# Autodesk Inventor assembly: Mini Stealthburner
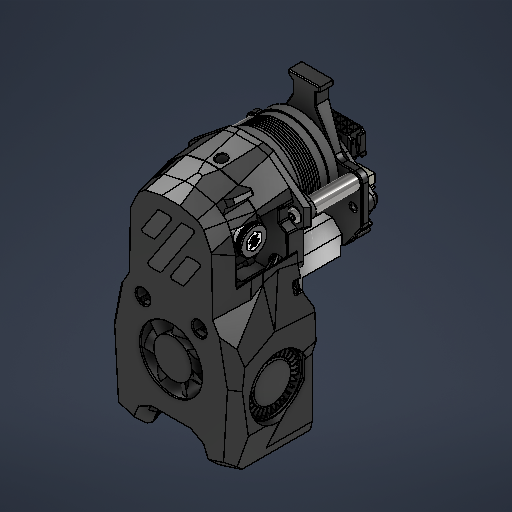
[picture p0: Inventor's stored thumbnail of the model, 512x512]
Saved by Autodesk Inventor 2026 (Build 300175050, 175E)
## iProperties
Created: 2025-05-09
Part Number: Mini Stealthburner
Document SubType Name: Assembly
Designer: AdminForWorker
Title: Mini Stealthburner
Author: AdminForWorker
## Documents named in this file (27)
- C:\Users\Joshua Eah\Documents\GitHub\Voron-0\CAD\Master Assembly\Toolhead\Mini Stealthburner.iam
- C:\Users\Joshua Eah\Documents\GitHub\Voron-0\CAD\Master Assembly\Toolhead\Parts\Extruder\36mm Round Stepper Motor.ipt
- C:\Users\Joshua Eah\Documents\GitHub\Voron-0\CAD\Master Assembly\Toolhead\Subassemblies\Hotend Assembly.iam
- C:\Users\Joshua Eah\Documents\GitHub\Voron-0\CAD\Master Assembly\Toolhead\Subassemblies\Front Cowling.iam
- C:\Users\Joshua Eah\Documents\GitHub\Voron-0\CAD\Machined Parts\X Carriage\X Carriage Body.ipt
- C:\Users\Joshua Eah\Documents\GitHub\Voron-0\CAD\Master Assembly\Hardware\M3x8 FHCS.ipt
- C:\Users\Joshua Eah\Documents\GitHub\Voron-0\CAD\Master Assembly\Hardware\M2x6 SHCS.ipt
- C:\Users\Joshua Eah\Documents\GitHub\Voron-0\CAD\Master Assembly\Hardware\M3x6 BHCS.ipt
- C:\Users\Joshua Eah\Documents\GitHub\Voron-0\CAD\Master Assembly\Hardware\M3x8 BHCS.ipt
- C:\Users\Joshua Eah\Documents\GitHub\Voron-0\CAD\Master Assembly\Hardware\M3x10 BHCS.ipt
- C:\Users\Joshua Eah\Documents\GitHub\Voron-0\CAD\Master Assembly\Hardware\M3x16 BHCS.ipt
- C:\Users\Joshua Eah\Documents\GitHub\Voron-0\CAD\Master Assembly\Hardware\M3x25 BHCS.ipt
- C:\Users\Joshua Eah\Documents\GitHub\Voron-0\CAD\Master Assembly\Hardware\M3x35 BHCS.ipt
- C:\Users\Joshua Eah\Documents\GitHub\Voron-0\CAD\Master Assembly\Hardware\Makerbeam T Nut.ipt
- C:\Users\Joshua Eah\Documents\GitHub\Voron-0\CAD\Master Assembly\Toolhead\Parts\Fans\3010 DC Axial Fan.ipt
- C:\Users\Joshua Eah\Documents\GitHub\Voron-0\CAD\Master Assembly\Toolhead\Parts\Fans\3010 DC Blower Fan.ipt
- C:\Users\Joshua Eah\Documents\GitHub\Voron-0\CAD\Master Assembly\Toolhead\Parts\Toolhead Frame\Latch.ipt
- C:\Users\Joshua Eah\Documents\GitHub\Voron-0\CAD\Master Assembly\Toolhead\Subassemblies\Tensioner Spring Assembly.iam
- C:\Users\Joshua Eah\Documents\GitHub\Voron-0\CAD\Master Assembly\Toolhead\Subassemblies\Idler Gear Assembly.iam
- C:\Users\Joshua Eah\Documents\GitHub\Voron-0\CAD\Master Assembly\Toolhead\Subassemblies\Drive Gear Assembly.iam
- C:\Users\Joshua Eah\Documents\GitHub\Voron-0\CAD\Master Assembly\Toolhead\Subassemblies\Guidler Assembly.iam
- C:\Users\Joshua Eah\Documents\GitHub\Voron-0\CAD\Master Assembly\Toolhead\Subassemblies\Extruder Midbody Assembly.iam
- C:\Users\Joshua Eah\Documents\GitHub\Voron-0\CAD\Master Assembly\Toolhead\Subassemblies\Shuttle.iam
- C:\Users\Joshua Eah\Documents\GitHub\Voron-0\CAD\Master Assembly\Toolhead\Subassemblies\Motor Plate Assembly.iam
- C:\Users\Joshua Eah\Documents\GitHub\Voron-0\CAD\Master Assembly\Toolhead\Parts\20mm M3 Spacer.ipt
- C:\Users\Joshua Eah\Documents\GitHub\Voron-0\CAD\Master Assembly\Toolhead\Parts\Toolhead Frame\V0.2_Toolhead_PCB_Mount.ipt
- C:\Users\Joshua Eah\Documents\GitHub\Voron-0\CAD\Master Assembly\Toolhead\Subassemblies\Toolhead_PCB.iam
## Components (46 placed, 26 different names)
1. Front Cowling:1 [sub-assembly] — Mate:5, Insert:4, Insert:11, Insert:12, Insert:13, Angle:1, Angle:2, Angle:3, Insert:16, Insert:17, Insert:18, Insert:19, Insert:29, Insert:30
2. Shuttle:1 [sub-assembly]
3. Tensioner Spring Assembly:1 [sub-assembly]
4. Latch:1 — Insert:4
5. Guidler Assembly:1 [sub-assembly]
6. Idler Gear Assembly:1 [sub-assembly] — Flush:1
7. Drive Gear Assembly:1 [sub-assembly] — Mate:5, Flush:1
8. Extruder Midbody Assembly:1 [sub-assembly] — Insert:5, Insert:6, Insert:7, Mate:9, Mate:10, Mate:11, Mate:12
9. M3x10 BHCS:1 — Insert:30
10. M3x10 BHCS:5 — Insert:29
11. M3x25 BHCS:1 — Insert:7
12. M3x25 BHCS:2 — Insert:5
13. M3x25 BHCS:3 — Insert:6
14. Motor Plate Assembly:1 [sub-assembly] — Insert:8, Insert:9, Insert:10, Mate:9, Mate:10, Mate:11, Insert:14, Insert:15, Mate:14
15. M3x6 BHCS:2 — Insert:9
16. M3x6 BHCS:3 — Insert:8
17. M3x10 BHCS:2 — Insert:10
18. 3010 DC Axial Fan:1 — Insert:13, Angle:3
19. 3010 DC Blower Fan:1 — Insert:11, Angle:1
20. 3010 DC Blower Fan:2 — Insert:12, Angle:2
21. 36mm Round Stepper Motor:1 — Insert:14, Mate:12, Mate:13, Insert:23, Insert:24
22. M3x10 BHCS:4 — Insert:15
23. M3x10 BHCS:3 — Mate:13, Mate:14
24. Hotend Assembly:1 [sub-assembly] — Insert:18, Insert:19, Insert:20, Insert:21
25. M3x35 BHCS:1 — Insert:17
26. M3x35 BHCS:2 — Insert:16
27. M3x16 BHCS:1 — Insert:22
28. 20mm M3 Spacer:1 — Insert:23, Mate:16
29. 20mm M3 Spacer:2 — Insert:24
30. X Carriage:1 — Insert:20, Insert:21, Insert:22, Insert:31, Insert:32, Insert:33, Insert:34, Insert:35, Insert:36, Insert:39, Insert:40
31. V0.2_Toolhead_PCB_Mount:1 — Insert:39, Insert:40, Mate:19, Mate:20, Mate:21, Insert:41, Insert:42, Insert:43, Insert:44
32. Toolhead_PCB:1 [sub-assembly] — Insert:43, Insert:44, Insert:45, Insert:46
33. M3x6 BHCS:5 — Insert:45
34. M3x6 BHCS:6 — Insert:46
35. M3x8 BHCS:1 — Insert:41
36. M3x8 BHCS:2 — Insert:42
37. M3x6 BHCS:1 — Mate:16, Mate:20
38. M3x6 BHCS:4 — Mate:19, Mate:21
39. M3x8 FHCS:1 — Insert:31, Insert:38
40. M3x8 FHCS:2 — Insert:32, Insert:37
41. M2x6 SHCS:1 — Insert:33
42. M2x6 SHCS:2 — Insert:35
43. M2x6 SHCS:3 — Insert:36
44. M2x6 SHCS:4 — Insert:34
45. Makerbeam T Nut:1 — Insert:37
46. Makerbeam T Nut:2 — Insert:38
## Relationships (63: Insert 41, Mate 18, Angle 3, Flush 1)
- [Mate]: Front Cowling:1 ↔ Shuttle:1
- [Mate]: Front Cowling:1 ↔ Shuttle:1
- [Insert]: Front Cowling:1 ↔ Guidler Assembly:1
- [Mate]: Tensioner Spring Assembly:1 ↔ Guidler Assembly:1
- [Mate]: Tensioner Spring Assembly:1 ↔ Guidler Assembly:1
- [Insert]: Guidler Assembly:1 ↔ Idler Gear Assembly:1
- Mate:5: Front Cowling:1 ↔ Drive Gear Assembly:1
- Flush:1: Idler Gear Assembly:1 ↔ Drive Gear Assembly:1
- Insert:4: Front Cowling:1 ↔ Latch:1
- [Mate]: Front Cowling:1 ↔ Extruder Midbody Assembly:1
- [Mate]: Front Cowling:1 ↔ Extruder Midbody Assembly:1
- [Mate]: Guidler Assembly:1 ↔ Extruder Midbody Assembly:1
- Insert:5: Extruder Midbody Assembly:1 ↔ M3x25 BHCS:2
- Insert:6: Extruder Midbody Assembly:1 ↔ M3x25 BHCS:3
- Insert:7: Extruder Midbody Assembly:1 ↔ M3x25 BHCS:1
- Insert:8: Motor Plate Assembly:1 ↔ M3x6 BHCS:3
- Insert:9: Motor Plate Assembly:1 ↔ M3x6 BHCS:2
- Insert:10: Motor Plate Assembly:1 ↔ M3x10 BHCS:2
- Mate:9: Extruder Midbody Assembly:1 ↔ Motor Plate Assembly:1
- Mate:10: Extruder Midbody Assembly:1 ↔ Motor Plate Assembly:1
- Mate:11: Extruder Midbody Assembly:1 ↔ Motor Plate Assembly:1
- Insert:11: Front Cowling:1 ↔ 3010 DC Blower Fan:1
- Insert:12: Front Cowling:1 ↔ 3010 DC Blower Fan:2
- Insert:13: Front Cowling:1 ↔ 3010 DC Axial Fan:1
- Angle:1 (0 deg): Front Cowling:1 ↔ 3010 DC Blower Fan:1
- Angle:2 (0 deg): Front Cowling:1 ↔ 3010 DC Blower Fan:2
- Angle:3 (0 deg): Front Cowling:1 ↔ 3010 DC Axial Fan:1
- Insert:14: Motor Plate Assembly:1 ↔ 36mm Round Stepper Motor:1
- Mate:12: Extruder Midbody Assembly:1 ↔ 36mm Round Stepper Motor:1
- Insert:15: Motor Plate Assembly:1 ↔ M3x10 BHCS:4
- Mate:13: 36mm Round Stepper Motor:1 ↔ M3x10 BHCS:3
- Mate:14: Motor Plate Assembly:1 ↔ M3x10 BHCS:3
- Insert:16: Front Cowling:1 ↔ M3x35 BHCS:2
- Insert:17: Front Cowling:1 ↔ M3x35 BHCS:1
- Insert:18: Front Cowling:1 ↔ Hotend Assembly:1
- Insert:19: Front Cowling:1 ↔ Hotend Assembly:1
- Insert:20: Hotend Assembly:1 ↔ X Carriage:1
- Insert:21: Hotend Assembly:1 ↔ X Carriage:1
- Insert:22: M3x16 BHCS:1 ↔ X Carriage:1
- Insert:23: 36mm Round Stepper Motor:1 ↔ 20mm M3 Spacer:1
- Insert:24: 36mm Round Stepper Motor:1 ↔ 20mm M3 Spacer:2
- Mate:16: 20mm M3 Spacer:1 ↔ M3x6 BHCS:1
- Insert:29: Front Cowling:1 ↔ M3x10 BHCS:5
- Insert:30: Front Cowling:1 ↔ M3x10 BHCS:1
- Insert:31: X Carriage:1 ↔ M3x8 FHCS:1
- Insert:32: X Carriage:1 ↔ M3x8 FHCS:2
- Insert:33: X Carriage:1 ↔ M2x6 SHCS:1
- Insert:34: X Carriage:1 ↔ M2x6 SHCS:4
- Insert:35: X Carriage:1 ↔ M2x6 SHCS:2
- Insert:36: X Carriage:1 ↔ M2x6 SHCS:3
- Insert:37: M3x8 FHCS:2 ↔ Makerbeam T Nut:1
- Insert:38: M3x8 FHCS:1 ↔ Makerbeam T Nut:2
- Insert:39: X Carriage:1 ↔ V0.2_Toolhead_PCB_Mount:1
- Insert:40: X Carriage:1 ↔ V0.2_Toolhead_PCB_Mount:1
- Mate:19: V0.2_Toolhead_PCB_Mount:1 ↔ M3x6 BHCS:4
- Mate:20: V0.2_Toolhead_PCB_Mount:1 ↔ M3x6 BHCS:1
- Mate:21: V0.2_Toolhead_PCB_Mount:1 ↔ M3x6 BHCS:4
- Insert:41: V0.2_Toolhead_PCB_Mount:1 ↔ M3x8 BHCS:1
- Insert:42: V0.2_Toolhead_PCB_Mount:1 ↔ M3x8 BHCS:2
- Insert:43: V0.2_Toolhead_PCB_Mount:1 ↔ Toolhead_PCB:1
- Insert:44: V0.2_Toolhead_PCB_Mount:1 ↔ Toolhead_PCB:1
- Insert:45: Toolhead_PCB:1 ↔ M3x6 BHCS:5
- Insert:46: Toolhead_PCB:1 ↔ M3x6 BHCS:6
